# Autodesk Inventor assembly: Assembly2
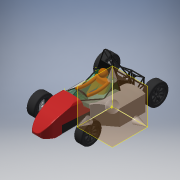
[picture p0: Inventor's stored thumbnail of the model, 180x180]
Saved by Autodesk Inventor 2018.1 (Build 221171000, 171)
## iProperties
Created: 2017-10-26
Part Number: Assembly2
Material: 一般
Document SubType Name: Assembly
Designer: KITformula
Author: KITformula
## Documents named in this file (3)
- Z:\各班フォルダ\2018\ボディ\カウル\AeroCAD2018\CAD\Inventor\Aero Parts\Side Pontoon\Assembly2.iam
- Z:\各班フォルダ\2018\ボディ\カウル\AeroCAD2018\CAD\Inventor\Aero Parts\Side Pontoon\part\ishispe.ipt
- Z:\各班フォルダ\2018\ボディ\カウル\AeroCAD2018\CAD\Inventor\Assembly(KS-14.ver)\KS-14_SLow\KS-14_SLow_replace.iam
## Components (2 placed, 2 different names)
1. ishispe:1 — フラッシュ:2, フラッシュ:3, フラッシュ:4
2. KS-14_SLow_replace:1 [sub-assembly] — メイト:4, メイト:5, メイト:6
## Relationships (6: Flush 3, Mate 3)
- フラッシュ:2 [Flush]: ishispe:1
- フラッシュ:3 [Flush]: ishispe:1
- フラッシュ:4 [Flush]: ishispe:1
- メイト:4 [Mate]: KS-14_SLow_replace:1
- メイト:5 [Mate]: KS-14_SLow_replace:1
- メイト:6 [Mate]: KS-14_SLow_replace:1
